# Autodesk Inventor assembly: dribbler
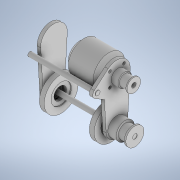
[picture p0: Inventor's stored thumbnail of the model, 180x180]
Saved by Autodesk Inventor 2020 (Build 240168000, 168)
## iProperties
Created: 2024-02-19
Part Number: dribbler
Document SubType Name: Assembly
Designer: 4s
Author: 4s
## Documents named in this file (10)
- C:\Users\4s\Documents\Inventor models\Asterisk\robot_v2\dribbler\dribbler.iam
- C:\Users\4s\Documents\Inventor models\Asterisk\robot_v2\dribbler\motor_sketch.ipt
- C:\Users\4s\Documents\Inventor models\Asterisk\robot_v2\dribbler\gear_16.ipt
- C:\Users\4s\Documents\Inventor models\Asterisk\robot_v2\dribbler\gear_20.ipt
- C:\Users\4s\Documents\Inventor models\Asterisk\robot_v2\dribbler\right_wall.ipt
- C:\Users\4s\Documents\Inventor models\Asterisk\robot_v2\dribbler\wheel.ipt
- C:\Users\4s\Documents\Inventor models\Asterisk\robot_v2\dribbler\roller.ipt
- C:\Users\4s\Documents\Inventor models\Asterisk\robot_v2\dribbler\left_wall.ipt
- C:\Users\4s\Documents\Inventor models\Asterisk\robot_v2\dribbler\sting_60.ipt
- C:\Users\4s\Documents\Inventor models\Asterisk\robot_v2\dribbler\sting_75.ipt
## Components (11 placed, 9 different names)
1. motor_sketch:1 — Совмещение:1, Совмещение:2, Совмещение:3, Совмещение:4, Совмещение:5, Угол:1, Совмещение:6, Совмещение:7, Совмещение:8, Совмещение:9
2. gear_16:1 — Совмещение:4, Совмещение:5
3. gear_20:1 — Угол:1, Совмещение:6, Совмещение:10
4. right_wall:1 — Совмещение:7, Совмещение:8, Совмещение:9, Совмещение:10, Совмещение:11, Совмещение:12, Совмещение:18, Заподлицо:1, Совмещение:20, Совмещение:24, Заподлицо:3
5. wheel:1 — Совмещение:11, Совмещение:12, Совмещение:17
6. wheel:2 — Совмещение:17, Совмещение:21, Совмещение:23
7. roller:1 — Совмещение:18, Заподлицо:1, Совмещение:19, Совмещение:25
8. roller:2 — Совмещение:22, Заподлицо:2, Заподлицо:4
9. left_wall:1 — Совмещение:19, Совмещение:20, Совмещение:21, Совмещение:22, Заподлицо:2, Совмещение:23
10. sting_60:1 — Совмещение:24, Заподлицо:3
11. sting_75:1 — Совмещение:25, Заподлицо:4
## Relationships (26: Mate 21, Flush 4, Angle 1)
- Совмещение:1 [Mate]: motor_sketch:1
- Совмещение:2 [Mate]: motor_sketch:1
- Совмещение:3 [Mate]: motor_sketch:1
- Совмещение:4 [Mate]: motor_sketch:1 ↔ gear_16:1
- Совмещение:5 [Mate] (4 mm): motor_sketch:1 ↔ gear_16:1
- Угол:1 [Angle] (180 deg): motor_sketch:1 ↔ gear_20:1
- Совмещение:6 [Mate] (3 mm): motor_sketch:1 ↔ gear_20:1
- Совмещение:7 [Mate]: motor_sketch:1 ↔ right_wall:1
- Совмещение:8 [Mate]: motor_sketch:1 ↔ right_wall:1
- Совмещение:9 [Mate]: motor_sketch:1 ↔ right_wall:1
- Совмещение:10 [Mate]: gear_20:1 ↔ right_wall:1
- Совмещение:11 [Mate]: right_wall:1 ↔ wheel:1
- Совмещение:12 [Mate] (3 mm): right_wall:1 ↔ wheel:1
- Совмещение:17 [Mate] (40 mm): wheel:1 ↔ wheel:2
- Совмещение:18 [Mate]: right_wall:1 ↔ roller:1
- Заподлицо:1 [Flush]: right_wall:1 ↔ roller:1
- Совмещение:19 [Mate]: roller:1 ↔ left_wall:1
- Совмещение:20 [Mate]: right_wall:1 ↔ left_wall:1
- Совмещение:21 [Mate]: wheel:2 ↔ left_wall:1
- Совмещение:22 [Mate]: roller:2 ↔ left_wall:1
- Заподлицо:2 [Flush]: roller:2 ↔ left_wall:1
- Совмещение:23 [Mate] (3 mm): wheel:2 ↔ left_wall:1
- Совмещение:24 [Mate]: right_wall:1 ↔ sting_60:1
- Заподлицо:3 [Flush] (-0.5 mm): right_wall:1 ↔ sting_60:1
- Совмещение:25 [Mate]: roller:1 ↔ sting_75:1
- Заподлицо:4 [Flush] (-0.5 mm): roller:2 ↔ sting_75:1
